# Autodesk Inventor assembly: Монтажная панель 19_11_2018
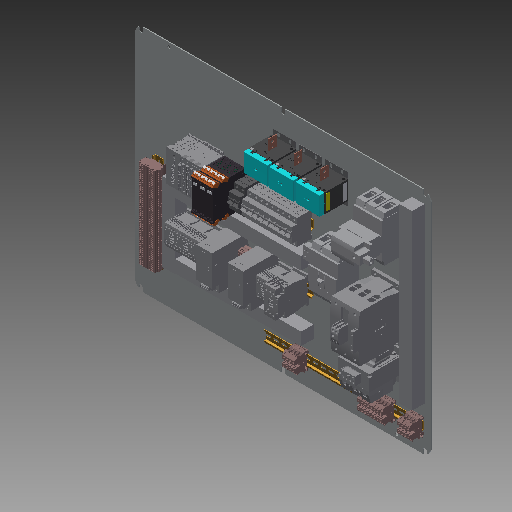
[picture p0: Inventor's stored thumbnail of the model, 512x512]
Saved by Autodesk Inventor 2019.3 (Build 233278000, 278)
## iProperties
Created: 2018-11-14
Part Number: Монтажная панель 19_11_2018
Material: Типовые
Document SubType Name: Assembly
Designer: A.Vlaschuk
Author: A.Vlaschuk
## Documents named in this file (31)
- E:\Work\01 Модернизация стенда гидроамортизаторов\КД\STAS60\Монтажная панель 19_11_2018.iam
- E:\Work\01 Модернизация стенда гидроамортизаторов\КД\STAS60\CAD Eaton\NZMB1-A100 (259079)\AIS2016\259079.iam
- E:\Work\01 Модернизация стенда гидроамортизаторов\КД\STAS60\CAD Eaton\NZMB1-A80 (259078)\AIS2016\259078.iam
- E:\Work\01 Модернизация стенда гидроамортизаторов\КД\STAS60\CAD Eaton\ZB150-70 (278463)\278463.ipt
- E:\Work\01 Модернизация стенда гидроамортизаторов\КД\STAS60\CAD Eaton\DILM80 (239402)\239416.ipt
- E:\Work\01 Модернизация стенда гидроамортизаторов\КД\STAS60\CAD Eaton\PL7-B25_2  (FAZ-B40_2)\278738.ipt
- E:\Work\01 Модернизация стенда гидроамортизаторов\КД\STAS60\CAD Eaton\PSG60F24RM (172882)\172882.ipt
- E:\Work\01 Модернизация стенда гидроамортизаторов\КД\STAS60\CAD Eaton\191080 XC-303-C32-002\191080.ipt
- E:\Work\01 Модернизация стенда гидроамортизаторов\КД\STAS60\CAD Eaton\179288 8AI-I\179288.ipt
- E:\Work\01 Модернизация стенда гидроамортизаторов\КД\STAS60\CAD Eaton\178771 8AIO-I\178791.ipt
- E:\Work\01 Модернизация стенда гидроамортизаторов\КД\STAS60\CAD Eaton\178790 8AO-U2\178790.ipt
- E:\Work\01 Модернизация стенда гидроамортизаторов\КД\STAS60\CAD Eaton\183180 16DIO-PC05\183180.ipt
- E:\Work\01 Модернизация стенда гидроамортизаторов\КД\STAS60\CAD Eaton\178772 4AI-PTNI\178772.ipt
- E:\Work\01 Модернизация стенда гидроамортизаторов\КД\STAS60\CAD Eaton\DILM38-10 (112442)\112442.ipt
- E:\Work\01 Модернизация стенда гидроамортизаторов\КД\STAS60\CAD Eaton\DILM12-10 (276845)\276845.ipt
- E:\Work\01 Модернизация стенда гидроамортизаторов\КД\STAS60\CAD Eaton\NZM1-XU208-240AC 259442\AIS2016\259434_part2.ipt
- E:\Work\01 Модернизация стенда гидроамортизаторов\КД\STAS60\Din Rail.ipt
- E:\Work\01 Модернизация стенда гидроамортизаторов\КД\STAS60\files-T2sV25yh1V\Т-0,66-1.iam
- E:\Work\01 Модернизация стенда гидроамортизаторов\КД\STAS60\CAD Eaton\DILM150-XH11_277946\277946.ipt
- E:\Work\01 Модернизация стенда гидроамортизаторов\КД\STAS60\CAD Eaton\PL7-B40_3 (FAZ-B40_3)\278851.ipt
- E:\Work\01 Модернизация стенда гидроамортизаторов\КД\STAS60\CAD Weidmuller Terminals\ZDU_2.5_1608510000\ZDU 2_5 1608510000.ipt
- E:\Work\01 Модернизация стенда гидроамортизаторов\КД\STAS60\CAD Weidmuller Terminals\WDU_10_1020300000\WDU 10 1020300000.ipt
- E:\Work\01 Модернизация стенда гидроамортизаторов\КД\STAS60\Din Rail_600.ipt
- E:\Work\01 Модернизация стенда гидроамортизаторов\КД\STAS60\RITTAL_USA_AE11305002\AIS2018\1100_02_16 (2).ipt
- E:\Work\01 Модернизация стенда гидроамортизаторов\КД\STAS60\Din Rail_200.ipt
- E:\Work\01 Модернизация стенда гидроамортизаторов\КД\STAS60\Кабельный канал 40х40х60.ipt
- E:\Work\01 Модернизация стенда гидроамортизаторов\КД\STAS60\CAD Weidmuller Terminals\WDU_10_1020300000\WDU 10 1020300000_КОПИЯ1.ipt
- E:\Work\01 Модернизация стенда гидроамортизаторов\КД\STAS60\WEIDMUELLER_SKDEMOCH20M221105600000\AIS2018\SK DEMO CH20M22 1105600000.iam
- E:\Work\01 Модернизация стенда гидроамортизаторов\КД\STAS60\Кабельный канал 40х40х400.ipt
- E:\Work\01 Модернизация стенда гидроамортизаторов\КД\STAS60\Кабельный канал 40х40х30.ipt
- E:\Work\01 Модернизация стенда гидроамортизаторов\КД\STAS60\CAD Eaton\NZM1-XS-R\AIS2018\100031_P3.ipt
## Components (118 placed, 28 different names)
1. 259079:1 [sub-assembly] — Совмещение:82, Совмещение:83, Совмещение:84, Совмещение:100, Заподлицо:12, Заподлицо:13
2. 259078:1 [sub-assembly] — Совмещение:90, Совмещение:91
3. 278463:1
4. 239416:1 — Заподлицо:3, Совмещение:85, Совмещение:86, Совмещение:87
5. 278738:1
6. 172882:1 — Совмещение:67, Совмещение:68
7. 172882:2
8. 191080:1 — Совмещение:79, Совмещение:80
9. 179288:1
10. 178791:1
11. 178790:1
12. 183180:1
13. 178772:1 — Совмещение:81
14. 112442:1
15. 276845:1
16. 259434_part2:1
17. DinRail:1 — Совмещение:50, Совмещение:51, Совмещение:77, Совмещение:78, Совмещение:79, Совмещение:80, Совмещение:81, Совмещение:92, Совмещение:93, Заподлицо:6
18. DinRail:3 — Совмещение:67, Совмещение:68, Совмещение:71, Совмещение:72, Заподлицо:7, Совмещение:95, Совмещение:96
19. Т-0,66-1:1 [sub-assembly] — Заподлицо:4
20. Т-0,66-1:2 [sub-assembly] — Заподлицо:4, Заподлицо:5
21. Т-0,66-1:3 [sub-assembly] — Заподлицо:5
22. 277946:1 — Заподлицо:3
23. DinRail:4 — Совмещение:55, Совмещение:59, Совмещение:60, Совмещение:69, Совмещение:70, Совмещение:73, Совмещение:74, Совмещение:88, Заподлицо:11
24. 1100_02_16 (2):1 — Совмещение:61, Совмещение:64, Совмещение:73, Совмещение:76, Совмещение:82, Совмещение:83, Совмещение:84, Совмещение:85, Совмещение:86, Совмещение:87, Совмещение:88, Совмещение:90, Совмещение:91, Совмещение:92, Совмещение:93, Заподлицо:6, Заподлицо:7, Совмещение:95, Совмещение:96, Заподлицо:8, Заподлицо:9, Совмещение:97, Совмещение:98, Заподлицо:10, Совмещение:99, Заподлицо:11, Заподлицо:13
25. DinRail:5 — Совмещение:61, Совмещение:62, Совмещение:63, Заподлицо:10, Совмещение:99
26. Кабельный канал 40х40х60:4 — Совмещение:64, Заподлицо:8
27. Кабельный канал 40х40х60:6 — Совмещение:76, Заподлицо:9
28. Кабельный канал 40х40х400:1 — Совмещение:97
29. Кабельный канал 40х40х30:1 — Совмещение:98
30. 100031_P3:1 — Совмещение:100, Заподлицо:12
31. 278851:1
32. 278851:2
33. 278851:3 — Совмещение:50, Совмещение:51
34. ZDU 2_5 1608510000:1
35. ZDU 2_5 1608510000:2
36. ZDU 2_5 1608510000:3
37. ZDU 2_5 1608510000:4
38. ZDU 2_5 1608510000:5
39. ZDU 2_5 1608510000:6
40. ZDU 2_5 1608510000:7
41. ZDU 2_5 1608510000:8 — Совмещение:71, Совмещение:72
42. WDU 10 1020300000:5 — Совмещение:59
43. WDU 10 1020300000:6
44. WDU 10 1020300000:7
45. WDU 10 1020300000:8 — Совмещение:60
46. ZDU 2_5 1608510000:9
47. ZDU 2_5 1608510000:10
48. ZDU 2_5 1608510000:11
49. ZDU 2_5 1608510000:12
50. ZDU 2_5 1608510000:13
51. ZDU 2_5 1608510000:14
52. ZDU 2_5 1608510000:15
53. ZDU 2_5 1608510000:16
54. ZDU 2_5 1608510000:17
55. ZDU 2_5 1608510000:18
56. ZDU 2_5 1608510000:19
57. ZDU 2_5 1608510000:20
58. ZDU 2_5 1608510000:21
59. ZDU 2_5 1608510000:22
60. ZDU 2_5 1608510000:23
61. ZDU 2_5 1608510000:24
62. ZDU 2_5 1608510000:25
63. ZDU 2_5 1608510000:26
64. ZDU 2_5 1608510000:27
65. ZDU 2_5 1608510000:28
66. ZDU 2_5 1608510000:29
67. ZDU 2_5 1608510000:30
68. ZDU 2_5 1608510000:31
69. ZDU 2_5 1608510000:32
70. ZDU 2_5 1608510000:33
71. ZDU 2_5 1608510000:34
72. ZDU 2_5 1608510000:35
73. ZDU 2_5 1608510000:36
74. ZDU 2_5 1608510000:37
75. ZDU 2_5 1608510000:38
76. ZDU 2_5 1608510000:39
77. ZDU 2_5 1608510000:40
78. ZDU 2_5 1608510000:41
79. ZDU 2_5 1608510000:42
80. ZDU 2_5 1608510000:43
81. ZDU 2_5 1608510000:44
82. ZDU 2_5 1608510000:45
83. ZDU 2_5 1608510000:46
84. ZDU 2_5 1608510000:47
85. ZDU 2_5 1608510000:48
86. ZDU 2_5 1608510000:49
87. ZDU 2_5 1608510000:50
88. ZDU 2_5 1608510000:51
89. ZDU 2_5 1608510000:52
90. ZDU 2_5 1608510000:53
91. ZDU 2_5 1608510000:54
92. ZDU 2_5 1608510000:55
93. ZDU 2_5 1608510000:56
94. ZDU 2_5 1608510000:57
95. ZDU 2_5 1608510000:58
96. ZDU 2_5 1608510000:59
97. ZDU 2_5 1608510000:60
98. ZDU 2_5 1608510000:61
99. ZDU 2_5 1608510000:62
100. ZDU 2_5 1608510000:63 — Совмещение:62, Совмещение:63
101. WDU 10 1020300000_КОПИЯ1:1
102. WDU 10 1020300000_КОПИЯ1:2
103. WDU 10 1020300000_КОПИЯ1:3
104. WDU 10 1020300000_КОПИЯ1:4 — Совмещение:69, Совмещение:70
105. WDU 10 1020300000:1 — Совмещение:55, Совмещение:74
106. WDU 10 1020300000:9
107. WDU 10 1020300000:10
108. WDU 10 1020300000:11
109. WDU 10 1020300000:12
110. WDU 10 1020300000:13
111. WDU 10 1020300000:14
112. WDU 10 1020300000:15
113. SK DEMO CH20M22 1105600000:1 [sub-assembly] — Совмещение:77, Совмещение:78
114. SK DEMO CH20M22 1105600000:2 [sub-assembly]
115. SK DEMO CH20M22 1105600000:3 [sub-assembly]
116. 276845:2
117. 276845:3
118. 276845:4
## Component patterns: (3 elements, first: 278851:1), (8 elements, first: ZDU 2_5 1608510000:1), (4 elements, first: WDU 10 1020300000:5), (55 elements, first: ZDU 2_5 1608510000:9), (4 elements, first: WDU 10 1020300000_КОПИЯ1:1), (8 elements, first: WDU 10 1020300000:1), (3 elements, first: SK DEMO CH20M22 1105600000:1), (3 elements, first: 276845:2)
## Relationships (82: Mate 71, Flush 11)
- [Mate]: 259078:1 ↔ 259434_part2:1
- [Mate]: 259078:1 ↔ 259434_part2:1
- [Mate]: 259078:1 ↔ 259434_part2:1
- [Mate]: 278463:1 ↔ 239416:1
- [Mate]: 278463:1 ↔ 239416:1
- [Mate]: 278463:1 ↔ 239416:1
- [Mate]: 191080:1 ↔ 179288:1
- [Mate]: 179288:1 ↔ 178791:1
- [Mate]: 178791:1 ↔ 178790:1
- [Mate]: 178790:1 ↔ 183180:1
- [Mate]: 183180:1 ↔ 178772:1
- [Mate]: 179288:1 ↔ 178791:1
- [Mate]: 178791:1 ↔ 178790:1
- [Mate]: 178790:1 ↔ 183180:1
- [Mate]: 183180:1 ↔ 178772:1
- [Mate]: 278738:1 ↔ DinRail:1
- [Mate]: 278738:1 ↔ DinRail:1
- [Mate]: 112442:1 ↔ DinRail:3
- [Mate]: 112442:1 ↔ DinRail:3
- [Mate]: 276845:1 ↔ DinRail:3
- [Mate]: 276845:1 ↔ DinRail:3
- [Mate]: DinRail:3 ↔ 276845:2
- [Mate]: DinRail:3 ↔ 276845:2
- [Mate]: 172882:2 ↔ DinRail:3
- [Mate]: 172882:2 ↔ DinRail:3
- [Mate] (5 mm): Т-0,66-1:1 ↔ Т-0,66-1:2
- [Mate] (5 mm): Т-0,66-1:2 ↔ Т-0,66-1:3
- [Mate]: 172882:2 ↔ DinRail:3
- [Mate]: 239416:1 ↔ 277946:1
- [Mate]: 239416:1 ↔ 277946:1
- [Mate]: 191080:1 ↔ 179288:1
- Заподлицо:3 [Flush]: 239416:1 ↔ 277946:1
- Заподлицо:4 [Flush]: Т-0,66-1:1 ↔ Т-0,66-1:2
- Заподлицо:5 [Flush]: Т-0,66-1:2 ↔ Т-0,66-1:3
- Совмещение:50 [Mate]: DinRail:1 ↔ 278851:3
- Совмещение:51 [Mate]: DinRail:1 ↔ 278851:3
- Совмещение:55 [Mate]: DinRail:4 ↔ WDU 10 1020300000:1
- Совмещение:59 [Mate]: DinRail:4 ↔ WDU 10 1020300000:5
- Совмещение:60 [Mate]: DinRail:4 ↔ WDU 10 1020300000:8
- Совмещение:61 [Mate]: 1100_02_16 (2):1 ↔ DinRail:5
- Совмещение:62 [Mate]: DinRail:5 ↔ ZDU 2_5 1608510000:63
- Совмещение:63 [Mate]: DinRail:5 ↔ ZDU 2_5 1608510000:63
- Совмещение:64 [Mate]: 1100_02_16 (2):1 ↔ Кабельный канал 40х40х60:4
- Совмещение:67 [Mate]: 172882:1 ↔ DinRail:3
- Совмещение:68 [Mate]: 172882:1 ↔ DinRail:3
- Совмещение:69 [Mate]: DinRail:4 ↔ WDU 10 1020300000_КОПИЯ1:4
- Совмещение:70 [Mate]: DinRail:4 ↔ WDU 10 1020300000_КОПИЯ1:4
- Совмещение:71 [Mate]: DinRail:3 ↔ ZDU 2_5 1608510000:8
- Совмещение:72 [Mate]: DinRail:3 ↔ ZDU 2_5 1608510000:8
- Совмещение:73 [Mate]: DinRail:4 ↔ 1100_02_16 (2):1
- Совмещение:74 [Mate]: DinRail:4 ↔ WDU 10 1020300000:1
- Совмещение:76 [Mate]: 1100_02_16 (2):1 ↔ Кабельный канал 40х40х60:6
- Совмещение:77 [Mate]: DinRail:1 ↔ SK DEMO CH20M22 1105600000:1
- Совмещение:78 [Mate]: DinRail:1 ↔ SK DEMO CH20M22 1105600000:1
- Совмещение:79 [Mate]: 191080:1 ↔ DinRail:1
- Совмещение:80 [Mate]: 191080:1 ↔ DinRail:1
- Совмещение:81 [Mate]: 178772:1 ↔ DinRail:1
- Совмещение:82 [Mate]: 259079:1 ↔ 1100_02_16 (2):1
- Совмещение:83 [Mate] (-150 mm): 259079:1 ↔ 1100_02_16 (2):1
- Совмещение:84 [Mate] (-80 mm): 259079:1 ↔ 1100_02_16 (2):1
- Совмещение:85 [Mate]: 239416:1 ↔ 1100_02_16 (2):1
- Совмещение:86 [Mate] (-100 mm): 239416:1 ↔ 1100_02_16 (2):1
- Совмещение:87 [Mate] (-300 mm): 239416:1 ↔ 1100_02_16 (2):1
- Совмещение:88 [Mate] (-80 mm): DinRail:4 ↔ 1100_02_16 (2):1
- Совмещение:90 [Mate] (-290 mm): 259078:1 ↔ 1100_02_16 (2):1
- Совмещение:91 [Mate] (-270 mm): 259078:1 ↔ 1100_02_16 (2):1
- Совмещение:92 [Mate]: DinRail:1 ↔ 1100_02_16 (2):1
- Совмещение:93 [Mate] (-270 mm): DinRail:1 ↔ 1100_02_16 (2):1
- Заподлицо:6 [Flush] (170 mm): DinRail:1 ↔ 1100_02_16 (2):1
- Заподлицо:7 [Flush] (170 mm): DinRail:3 ↔ 1100_02_16 (2):1
- Совмещение:95 [Mate]: DinRail:3 ↔ 1100_02_16 (2):1
- Совмещение:96 [Mate] (-455 mm): DinRail:3 ↔ 1100_02_16 (2):1
- Заподлицо:8 [Flush] (170 mm): 1100_02_16 (2):1 ↔ Кабельный канал 40х40х60:4
- Заподлицо:9 [Flush] (170 mm): 1100_02_16 (2):1 ↔ Кабельный канал 40х40х60:6
- Совмещение:97 [Mate]: 1100_02_16 (2):1 ↔ Кабельный канал 40х40х400:1
- Совмещение:98 [Mate]: 1100_02_16 (2):1 ↔ Кабельный канал 40х40х30:1
- Заподлицо:10 [Flush] (100 mm): 1100_02_16 (2):1 ↔ DinRail:5
- Совмещение:99 [Mate] (-80 mm): 1100_02_16 (2):1 ↔ DinRail:5
- Заподлицо:11 [Flush] (420 mm): DinRail:4 ↔ 1100_02_16 (2):1
- Совмещение:100 [Mate]: 259079:1 ↔ 100031_P3:1
- Заподлицо:12 [Flush]: 259079:1 ↔ 100031_P3:1
- Заподлицо:13 [Flush] (90 mm): 259079:1 ↔ 1100_02_16 (2):1
